# Autodesk Inventor assembly: Hoverboard-Robot
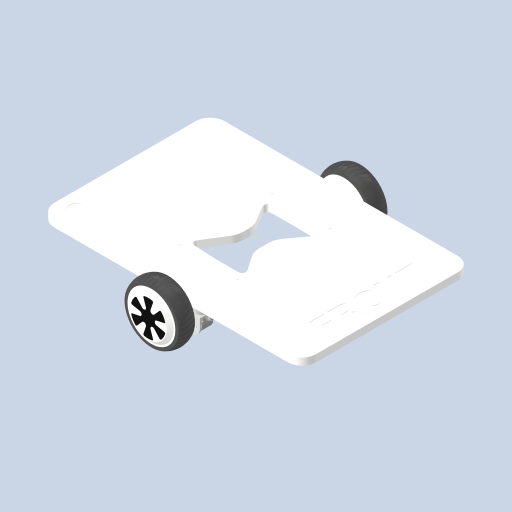
[picture p0: Inventor's stored thumbnail of the model, 512x512]
Saved by Autodesk Inventor 2023 (Build 270158000, 158)
## iProperties
Created: 2022-11-10
Part Number: Hoverboard-Robot
Document SubType Name: Assembly
Designer: haash
Author: haash
## Documents named in this file (9)
- C:\Users\haash\OneDrive\Documents\Projects\Hoverboard-Robot\Hoverboard-Robot.iam
- C:\Users\haash\OneDrive\Documents\Projects\Hoverboard-Robot\BaseBoard.ipt
- C:\Users\haash\OneDrive\Documents\Projects\Hoverboard-Robot\Center-Cover.ipt
- C:\Users\haash\OneDrive\Documents\Projects\Hoverboard-Robot\DriveWheelAssembly.iam
- C:\Users\haash\OneDrive\Documents\Projects\Hoverboard-Robot\DriveWheelAssembly_MIR.iam
- C:\Users\haash\OneDrive\Documents\Projects\Hoverboard-Robot\Batteries\5S2P_Battery_Pack.iam
- C:\Users\haash\OneDrive\Documents\Projects\Hoverboard-Robot\Batteries\H7-12FR_Battery.ipt
- C:\Users\haash\OneDrive\Documents\Projects\Hoverboard-Robot\Batteries\5S2P-Holder.ipt
- C:\Users\haash\OneDrive\Documents\Projects\Hoverboard-Robot\Batteries\H7-12FR_Holder.ipt
## Components (9 placed, 8 different names)
1. BaseBoard:1 — Flush:4, Flush:5, Flush:6, Flush:7, Mate:35, Mate:39, Angle:3
2. Center-Cover:1 — Flush:4, Flush:8, Mate:34
3. DriveWheelAssembly:1 [sub-assembly]
4. DriveWheelAssembly_MIR:1 [sub-assembly]
5. 5S2P_Battery_Pack:1 [sub-assembly] — Mate:36, Mate:38, Flush:9
6. H7-12FR_Battery:1 — Mate:40, Mate:41, Mate:42
7. 5S2P_Battery_Pack:2 [sub-assembly] — Mate:37, Mate:38, Flush:9
8. 5S2P-Holder:1 — Mate:35, Mate:36, Mate:37
9. H7-12FR_Holder:1 — Mate:39, Mate:40, Angle:3, Mate:41, Mate:42
## Relationships (24: Mate 15, Flush 7, Angle 2)
- [Mate]: BaseBoard:1 ↔ DriveWheelAssembly:1
- [Mate]: BaseBoard:1 ↔ DriveWheelAssembly:1
- [Mate] (-25 mm): BaseBoard:1 ↔ DriveWheelAssembly:1
- [Mate] (-25 mm): BaseBoard:1 ↔ DriveWheelAssembly:1
- [Mate] (47 mm): BaseBoard:1 ↔ DriveWheelAssembly:1
- [Angle] (0 deg): BaseBoard:1 ↔ DriveWheelAssembly:1
- [Flush] (-16.25 mm): BaseBoard:1 ↔ DriveWheelAssembly:1
- [Mate] (-2 mm): BaseBoard:1 ↔ DriveWheelAssembly:1
- Flush:4: BaseBoard:1 ↔ Center-Cover:1
- Flush:5: BaseBoard:1
- Flush:6: BaseBoard:1
- Flush:7: BaseBoard:1
- Flush:8: Center-Cover:1
- Mate:34: Center-Cover:1
- Mate:35: BaseBoard:1 ↔ 5S2P-Holder:1
- Mate:36: 5S2P_Battery_Pack:1 ↔ 5S2P-Holder:1
- Mate:37: 5S2P_Battery_Pack:2 ↔ 5S2P-Holder:1
- Mate:38: 5S2P_Battery_Pack:1 ↔ 5S2P_Battery_Pack:2
- Flush:9: 5S2P_Battery_Pack:1 ↔ 5S2P_Battery_Pack:2
- Mate:39: BaseBoard:1 ↔ H7-12FR_Holder:1
- Mate:40: H7-12FR_Battery:1 ↔ H7-12FR_Holder:1
- Angle:3 (0 deg): BaseBoard:1 ↔ H7-12FR_Holder:1
- Mate:41: H7-12FR_Battery:1 ↔ H7-12FR_Holder:1
- Mate:42: H7-12FR_Battery:1 ↔ H7-12FR_Holder:1
